# Autodesk Inventor assembly: Сборка xfcnm
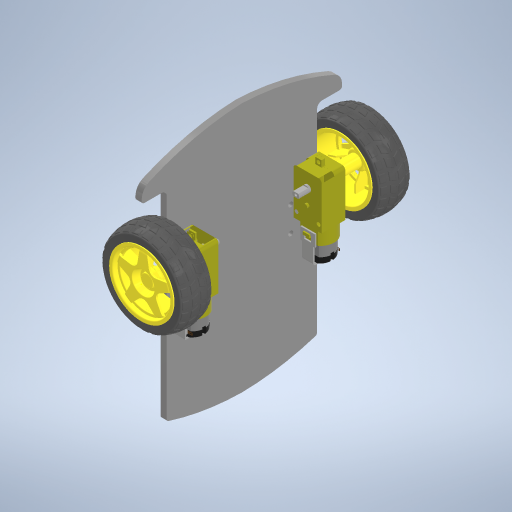
[picture p0: Inventor's stored thumbnail of the model, 512x512]
Saved by Autodesk Inventor 2023 (Build 270158000, 158)
## iProperties
Created: 2023-11-16
Part Number: Сборка xfcnm
Document SubType Name: Assembly
Designer: gando
Author: gando
## Documents named in this file (7)
- C:\Users\gando\OneDrive\Документы\Сборка xfcnm.iam
- C:\Users\gando\OneDrive\Документы\Основа платформы.ipt
- C:\Users\gando\OneDrive\Рабочий стол\Колёсик\wheel-d65x25-1.snapshot.5\Wheel D65x25.ipt
- C:\Users\gando\OneDrive\Рабочий стол\СТЛ моторчик\Imported Components\Motor Reducer For Arduino\Motor Reducer For Arduino.ipt
- C:\Users\gando\OneDrive\Рабочий стол\СТЛ моторчик\Imported Components\Motor Reducer For Arduino\Motor Reducer For Arduino_MIR.ipt
- C:\Users\gando\OneDrive\Рабочий стол\СТЛ моторчик\Imported Components\Motor Reducer For Arduino\Motor Reducer For Arduino_CPY.ipt
- C:\Users\gando\OneDrive\Рабочий стол\Колёсик\wheel-d65x25-1.snapshot.5\Wheel D65x25_CPY1.ipt
## Components (6 placed, 6 different names)
1. Основа платформы:1 — Совмещение:1, Заподлицо:1, Совмещение:2, Совмещение:3, Заподлицо:3
2. Wheel D65x25:1 — Вставка:1
3. Motor Reducer For Arduino:1 — Совмещение:1, Заподлицо:1, Совмещение:2, Вставка:1, Заподлицо:2
4. Motor Reducer For Arduino_MIR:1
5. Motor Reducer For Arduino_CPY:1 — Совмещение:3, Заподлицо:2, Заподлицо:3, Вставка:2
6. Wheel D65x25_CPY1:1 — Вставка:2
## Relationships (8: Mate 3, Flush 3, Insert 2)
- Совмещение:1 [Mate]: Основа платформы:1 ↔ Motor Reducer For Arduino:1
- Заподлицо:1 [Flush]: Основа платформы:1 ↔ Motor Reducer For Arduino:1
- Совмещение:2 [Mate] (32.5 mm): Основа платформы:1 ↔ Motor Reducer For Arduino:1
- Вставка:1 [Insert]: Wheel D65x25:1 ↔ Motor Reducer For Arduino:1
- Совмещение:3 [Mate]: Основа платформы:1 ↔ Motor Reducer For Arduino_CPY:1
- Заподлицо:2 [Flush]: Motor Reducer For Arduino:1 ↔ Motor Reducer For Arduino_CPY:1
- Заподлицо:3 [Flush]: Основа платформы:1 ↔ Motor Reducer For Arduino_CPY:1
- Вставка:2 [Insert]: Motor Reducer For Arduino_CPY:1 ↔ Wheel D65x25_CPY1:1
